# Autodesk Inventor assembly: Drehgreifer
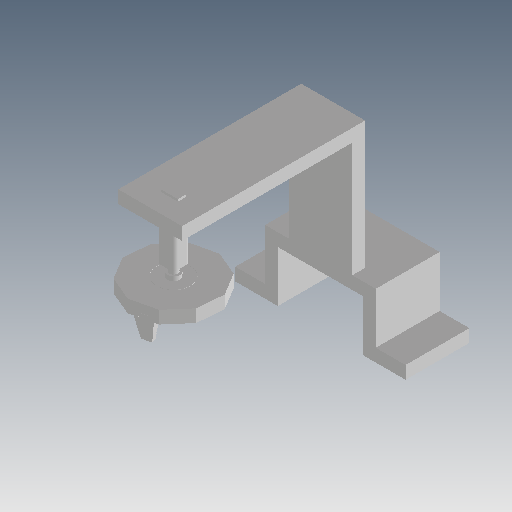
[picture p0: Inventor's stored thumbnail of the model, 512x512]
Saved by Autodesk Inventor 2020 (Build 240168000, 168)
## iProperties
Created: 2020-03-18
Part Number: Drehgreifer
Document SubType Name: Assembly
Designer: franz
Author: franz
## Documents named in this file (7)
- E:\Privat\Projekte\SPS_Training\Unity_SPS_Simulation\Unity_SPS_Schrittkette\CAD\Foerderband_V1\Drehgreifer\Drehgreifer.iam
- E:\Privat\Projekte\SPS_Training\Unity_SPS_Simulation\Unity_SPS_Schrittkette\CAD\Foerderband_V1\Drehgreifer\Staender.ipt
- E:\Privat\Projekte\SPS_Training\Unity_SPS_Simulation\Unity_SPS_Schrittkette\CAD\Foerderband_V1\Drehgreifer\Hubvorrichtung.ipt
- E:\Privat\Projekte\SPS_Training\Unity_SPS_Simulation\Unity_SPS_Schrittkette\CAD\Foerderband_V1\Drehgreifer\Hubstange.ipt
- E:\Privat\Projekte\SPS_Training\Unity_SPS_Simulation\Unity_SPS_Schrittkette\CAD\Foerderband_V1\Drehgreifer\Oberteil.ipt
- E:\Privat\Projekte\SPS_Training\Unity_SPS_Simulation\Unity_SPS_Schrittkette\CAD\Foerderband_V1\Drehgreifer\Unterteil.ipt
- E:\Privat\Projekte\SPS_Training\Unity_SPS_Simulation\Unity_SPS_Schrittkette\CAD\Foerderband_V1\Drehgreifer\Finger.ipt
## Components (7 placed, 6 different names)
1. Staender:1 — Starr:1
2. Hubvorrichtung:1 — Starr:1, Zylindrisch:1, Winkel:1
3. Hubstange:1 — Zylindrisch:1, Winkel:1, Starr:2
4. Oberteil:1 — Starr:2, Drehbar:1
5. Unterteil:1 — Drehbar:1, Passend:1, Passend:2, Passend:3, Passend:4, Zylindrisch:2, Zylindrisch:3
6. Finger:1 — Passend:2, Passend:3, Zylindrisch:3
7. Finger:2 — Passend:1, Passend:4, Zylindrisch:2
## Relationships (11: Mate 4, CylindricalJoint 3, WeldJoint 2, Angle 1, RevoluteJoint 1)
- Starr:1 [WeldJoint]: Staender:1 ↔ Hubvorrichtung:1
- Zylindrisch:1 [CylindricalJoint]: Hubvorrichtung:1 ↔ Hubstange:1
- Winkel:1 [Angle] (0 deg): Hubvorrichtung:1 ↔ Hubstange:1
- Starr:2 [WeldJoint]: Hubstange:1 ↔ Oberteil:1
- Drehbar:1 [RevoluteJoint]: Oberteil:1 ↔ Unterteil:1
- Passend:1 [Mate]: Unterteil:1 ↔ Finger:2
- Passend:2 [Mate]: Unterteil:1 ↔ Finger:1
- Passend:3 [Mate]: Unterteil:1 ↔ Finger:1
- Passend:4 [Mate]: Unterteil:1 ↔ Finger:2
- Zylindrisch:2 [CylindricalJoint]: Unterteil:1 ↔ Finger:2
- Zylindrisch:3 [CylindricalJoint]: Unterteil:1 ↔ Finger:1
